# Autodesk Inventor assembly: final stand
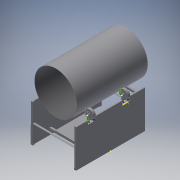
[picture p0: Inventor's stored thumbnail of the model, 180x180]
Saved by Autodesk Inventor 2019 (Build 230136000, 136)
## iProperties
Created: 2020-02-15
Part Number: final stand
Document SubType Name: Assembly
Designer: Admin
Author: Admin
## Documents named in this file (4)
- C:\Users\admin\Desktop\Exploration\final stand.iam
- C:\Users\admin\Desktop\Exploration\stand2.0.ipt
- C:\Users\admin\Desktop\Exploration\roller complete.iam
- C:\Users\admin\Desktop\Exploration\Finally_we_are_done_with_drum.ipt
## Components (6 placed, 3 different names)
1. stand2.0:1 — Rigid:1, Rigid:2, Rigid:3, Rigid:4
2. roller complete:1 [sub-assembly] — Rigid:1, Tangent:5, Tangent:12
3. roller complete:2 [sub-assembly] — Rigid:2, Tangent:1, Tangent:3, Tangent:4, Tangent:11
4. roller complete:3 [sub-assembly] — Rigid:3, Tangent:6, Tangent:9
5. roller complete:4 [sub-assembly] — Rigid:4, Tangent:2, Tangent:7, Tangent:8, Tangent:10
6. Finally_we_are_done_with_drum:1 — Tangent:1, Tangent:2, Tangent:3, Tangent:4, Tangent:5, Tangent:6, Tangent:7, Tangent:8, Tangent:9, Tangent:10, Tangent:11, Tangent:12
## Relationships (16: Tangent 12, WeldJoint 4)
- Rigid:1 [WeldJoint]: stand2.0:1 ↔ roller complete:1
- Rigid:2 [WeldJoint]: stand2.0:1 ↔ roller complete:2
- Rigid:3 [WeldJoint]: stand2.0:1 ↔ roller complete:3
- Rigid:4 [WeldJoint]: stand2.0:1 ↔ roller complete:4
- Tangent:1: roller complete:2 ↔ Finally_we_are_done_with_drum:1
- Tangent:2: roller complete:4 ↔ Finally_we_are_done_with_drum:1
- Tangent:3: roller complete:2 ↔ Finally_we_are_done_with_drum:1
- Tangent:4: roller complete:2 ↔ Finally_we_are_done_with_drum:1
- Tangent:5: roller complete:1 ↔ Finally_we_are_done_with_drum:1
- Tangent:6: roller complete:3 ↔ Finally_we_are_done_with_drum:1
- Tangent:7: roller complete:4 ↔ Finally_we_are_done_with_drum:1
- Tangent:8: roller complete:4 ↔ Finally_we_are_done_with_drum:1
- Tangent:9: roller complete:3 ↔ Finally_we_are_done_with_drum:1
- Tangent:10: roller complete:4 ↔ Finally_we_are_done_with_drum:1
- Tangent:11: roller complete:2 ↔ Finally_we_are_done_with_drum:1
- Tangent:12: roller complete:1 ↔ Finally_we_are_done_with_drum:1
